# Autodesk Inventor assembly: DelrinWheel_MIR
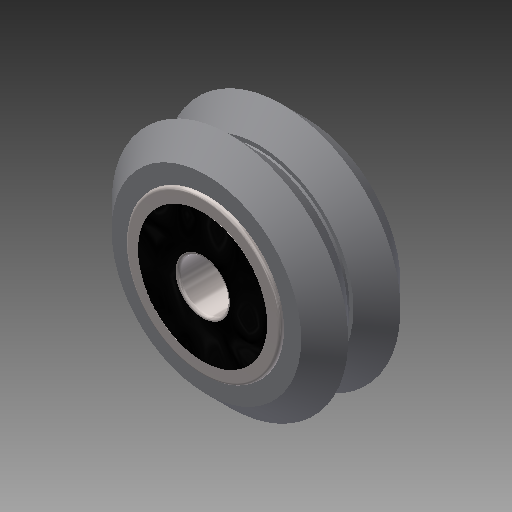
[picture p0: Inventor's stored thumbnail of the model, 512x512]
Saved by Autodesk Inventor 2017 (Build 210142000, 142)
## iProperties
Created: 2016-07-20
Part Number: DelrinWheel_MIR
Document SubType Name: Assembly
Designer: User
Author: User
## Documents named in this file (4)
- C:\All INVENTOR\SL-Inventor\SL-Beast 3D Printer\DelrinWheel_MIR.iam
- C:\All INVENTOR\SL-Inventor\SL-Beast 3D Printer\dELRIN_MIR1.ipt
- C:\All INVENTOR\SL-Inventor\SL-Beast 3D Printer\SKF 625_MIR1.ipt
- C:\All INVENTOR\SL-Inventor\SL-Beast 3D Printer\SKF 625_CPY_MIR1.ipt
## Components (3 placed, 3 different names)
1. dELRIN_MIR1:1 — Mate:2, Mate:1, Mate:4, Mate:3
2. SKF 625_MIR1:1 — Mate:2, Mate:1
3. SKF 625_CPY_MIR1:1 — Mate:4, Mate:3
## Relationships (4: Mate 4)
- Mate:2: dELRIN_MIR1:1 ↔ SKF 625_MIR1:1
- Mate:1: dELRIN_MIR1:1 ↔ SKF 625_MIR1:1
- Mate:4: dELRIN_MIR1:1 ↔ SKF 625_CPY_MIR1:1
- Mate:3: dELRIN_MIR1:1 ↔ SKF 625_CPY_MIR1:1
